# Autodesk Inventor assembly: Chess board
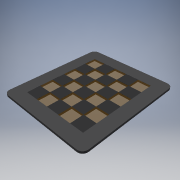
[picture p0: Inventor's stored thumbnail of the model, 180x180]
Saved by Autodesk Inventor 2016 (Build 200138000, 138)
## iProperties
Created: 2015-08-29
Part Number: Chess board
Document SubType Name: Assembly
Designer: Pranav
Author: Pranav
## Documents named in this file (4)
- D:\Users\Pranav\Documents\Junior Design Models\Chess board.iam
- D:\Users\Pranav\Documents\Junior Design Models\Tile.ipt
- D:\Users\Pranav\Documents\Junior Design Models\Tile2.ipt
- D:\Users\Pranav\Documents\Junior Design Models\Border.ipt
## Components (31 placed, 3 different names)
1. Tile:1 — Mate:2, Flush:1, Flush:2, Flush:3, Flush:13, Mate:4, Flush:15
2. Tile:2 — Flush:3, Flush:4, Flush:5, Flush:16, Mate:7, Mate:8, Flush:17, Flush:28, Mate:26, Mate:44
3. Tile:3 — Mate:1, Flush:2, Flush:8, Flush:12, Mate:9, Flush:18
4. Tile:4 — Flush:9, Flush:14, Mate:3, Mate:11, Flush:20, Mate:17
5. Tile:5 — Flush:8, Mate:5, Mate:6, Mate:12, Flush:21, Mate:21
6. Tile:6 — Flush:7, Mate:10, Flush:19
7. Tile2:1 — Mate:1, Mate:2, Flush:1, Flush:9, Flush:12, Flush:13, Flush:14, Mate:3, Mate:5
8. Tile2:2 — Flush:4, Mate:8, Flush:17, Flush:47
9. Tile2:3 — Flush:5, Flush:6, Mate:4, Flush:15, Mate:6, Flush:16, Mate:7, Mate:23
10. Tile2:4 — Flush:6, Flush:7, Flush:10, Mate:12, Flush:21, Flush:24, Flush:25, Flush:26, Mate:15, Flush:27, Mate:16
11. Tile2:5 — Flush:10, Flush:11, Mate:9, Flush:18, Mate:10, Flush:19, Mate:45
12. Tile2:6 — Flush:11, Mate:11, Flush:20, Flush:22, Flush:23, Mate:13
13. Tile:7 — Flush:28, Flush:29, Flush:31, Mate:39, Mate:40, Mate:43, Flush:45, Flush:46
14. Tile:8 — Flush:26, Mate:15, Flush:27, Mate:19, Flush:35, Flush:36, Mate:22, Mate:29
15. Tile:9 — Flush:29, Flush:30, Flush:42, Mate:31, Mate:36, Flush:43
16. Tile:10 — Flush:31, Flush:32, Flush:38, Mate:27, Mate:28, Flush:39, Mate:30, Flush:40, Flush:41
17. Tile:11 — Flush:30, Mate:41, Mate:42
18. Tile:12 — Flush:32, Flush:33, Mate:32, Mate:33, Mate:34, Mate:38
19. Tile:13 — Flush:22, Flush:23, Mate:13, Mate:18
20. Tile:14 — Flush:24, Flush:25, Mate:16, Flush:34, Mate:20
21. Tile:15 — Flush:33, Mate:23, Mate:24, Mate:25, Flush:37, Mate:37, Flush:44
22. Tile2:7 — Flush:34, Mate:17, Mate:18
23. Tile2:8 — Mate:19, Mate:20, Flush:35, Flush:38, Mate:27
24. Tile2:9 — Mate:21, Flush:36, Mate:22, Mate:24, Mate:32
25. Tile2:10 — Mate:34, Mate:36, Flush:43, Mate:42
26. Tile2:11 — Mate:37, Flush:44, Mate:38, Mate:40, Mate:41
27. Tile2:12 — Mate:25, Mate:26, Flush:37, Mate:39
28. Tile2:13 — Mate:43, Flush:45, Flush:46
29. Tile2:14 — Mate:28, Flush:39, Mate:29, Mate:33
30. Tile2:15 — Mate:30, Flush:40, Flush:41, Flush:42, Mate:31
31. Border:1 — Mate:44, Mate:45, Flush:47
## Relationships (90: Flush 47, Mate 43)
- Mate:1: Tile:3 ↔ Tile2:1
- Mate:2: Tile:1 ↔ Tile2:1
- Flush:1: Tile:1 ↔ Tile2:1
- Flush:2: Tile:1 ↔ Tile:3
- Flush:3: Tile:1 ↔ Tile:2
- Flush:4: Tile:2 ↔ Tile2:2
- Flush:5: Tile:2 ↔ Tile2:3
- Flush:6: Tile2:3 ↔ Tile2:4
- Flush:7: Tile:6 ↔ Tile2:4
- Flush:8: Tile:3 ↔ Tile:5
- Flush:9: Tile:4 ↔ Tile2:1
- Flush:10: Tile2:4 ↔ Tile2:5
- Flush:11: Tile2:5 ↔ Tile2:6
- Flush:12: Tile:3 ↔ Tile2:1
- Flush:13: Tile:1 ↔ Tile2:1
- Flush:14: Tile:4 ↔ Tile2:1
- Mate:3: Tile:4 ↔ Tile2:1
- Mate:4: Tile:1 ↔ Tile2:3
- Flush:15: Tile:1 ↔ Tile2:3
- Mate:5: Tile:5 ↔ Tile2:1
- Mate:6: Tile:5 ↔ Tile2:3
- Flush:16: Tile:2 ↔ Tile2:3
- Mate:7: Tile:2 ↔ Tile2:3
- Mate:8: Tile:2 ↔ Tile2:2
- Flush:17: Tile:2 ↔ Tile2:2
- Mate:9: Tile:3 ↔ Tile2:5
- Flush:18: Tile:3 ↔ Tile2:5
- Mate:10: Tile:6 ↔ Tile2:5
- Flush:19: Tile:6 ↔ Tile2:5
- Mate:11: Tile:4 ↔ Tile2:6
- Flush:20: Tile:4 ↔ Tile2:6
- Mate:12: Tile:5 ↔ Tile2:4
- Flush:21: Tile:5 ↔ Tile2:4
- Flush:22: Tile2:6 ↔ Tile:13
- Flush:23: Tile2:6 ↔ Tile:13
- Mate:13: Tile2:6 ↔ Tile:13
- Flush:24: Tile2:4 ↔ Tile:14
- Flush:25: Tile2:4 ↔ Tile:14
- Flush:26: Tile2:4 ↔ Tile:8
- Mate:15: Tile2:4 ↔ Tile:8
- Flush:27: Tile2:4 ↔ Tile:8
- Mate:16: Tile2:4 ↔ Tile:14
- Flush:28: Tile:2 ↔ Tile:7
- Flush:29: Tile:7 ↔ Tile:9
- Flush:30: Tile:9 ↔ Tile:11
- Flush:31: Tile:7 ↔ Tile:10
- Flush:32: Tile:10 ↔ Tile:12
- Flush:33: Tile:12 ↔ Tile:15
- Flush:34: Tile:14 ↔ Tile2:7
- Mate:17: Tile:4 ↔ Tile2:7
- Mate:18: Tile:13 ↔ Tile2:7
- Mate:19: Tile:8 ↔ Tile2:8
- Mate:20: Tile:14 ↔ Tile2:8
- Flush:35: Tile:8 ↔ Tile2:8
- Mate:21: Tile:5 ↔ Tile2:9
- Flush:36: Tile:8 ↔ Tile2:9
- Mate:22: Tile:8 ↔ Tile2:9
- Mate:23: Tile2:3 ↔ Tile:15
- Mate:24: Tile:15 ↔ Tile2:9
- Mate:25: Tile:15 ↔ Tile2:12
- Mate:26: Tile:2 ↔ Tile2:12
- Flush:37: Tile:15 ↔ Tile2:12
- Flush:38: Tile:10 ↔ Tile2:8
- Mate:27: Tile:10 ↔ Tile2:8
- Mate:28: Tile:10 ↔ Tile2:14
- Flush:39: Tile:10 ↔ Tile2:14
- Mate:29: Tile:8 ↔ Tile2:14
- Mate:30: Tile:10 ↔ Tile2:15
- Flush:40: Tile:10 ↔ Tile2:15
- Flush:41: Tile:10 ↔ Tile2:15
- Flush:42: Tile:9 ↔ Tile2:15
- Mate:31: Tile:9 ↔ Tile2:15
- Mate:32: Tile:12 ↔ Tile2:9
- Mate:33: Tile:12 ↔ Tile2:14
- Mate:34: Tile:12 ↔ Tile2:10
- Mate:36: Tile:9 ↔ Tile2:10
- Flush:43: Tile:9 ↔ Tile2:10
- Mate:37: Tile:15 ↔ Tile2:11
- Flush:44: Tile:15 ↔ Tile2:11
- Mate:38: Tile:12 ↔ Tile2:11
- Mate:39: Tile:7 ↔ Tile2:12
- Mate:40: Tile:7 ↔ Tile2:11
- Mate:41: Tile:11 ↔ Tile2:11
- Mate:42: Tile:11 ↔ Tile2:10
- Mate:43: Tile:7 ↔ Tile2:13
- Flush:45: Tile:7 ↔ Tile2:13
- Flush:46: Tile:7 ↔ Tile2:13
- Mate:44: Tile:2 ↔ Border:1
- Mate:45: Tile2:5 ↔ Border:1
- Flush:47: Tile2:2 ↔ Border:1
